# Autodesk Inventor assembly: DriveTrainAssembly
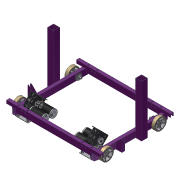
[picture p0: Inventor's stored thumbnail of the model, 180x180]
Saved by Autodesk Inventor 2012 (Build 160160000, 160)
## iProperties
Created: 2013-01-06
Part Number: DriveTrainAssembly
Document SubType Name: Assembly
Designer: JesseK
Mass: 18854.9 g
Surface Area: 24329.7 cm^2
Volume: 23563.9 cm^3
Density: 0.800159 g/cm^3
Author: JesseK
## Documents named in this file (15)
- Z:\UserData\Documents\Inventor\team1885frc\Robot2013\DriveTrain\DriveTrainAssembly.iam
- Z:\UserData\Documents\Inventor\team1885frc\Robot2013\DriveTrain\DriveTrainFrameAssembly.iam
- Z:\UserData\Documents\Inventor\team1885frc\Robot2013\DriveTrain\WheelBearingBlock.ipt
- Z:\UserData\Documents\Inventor\team1885frc\Hardware\Bearings\500id_1.125od_hex_flange_bearing.ipt
- Z:\UserData\Documents\Inventor\team1885frc\Robot2013\DriveTrain\WheelAxle.ipt
- Z:\UserData\Documents\Inventor\team1885frc\AndyMark\4 Perf ThruTread 500 Hex.ipt
- Z:\UserData\Documents\Inventor\team1885frc\VEXPro\Gears\44T-0500-hex.217-2710.20121204.ipt
- Z:\UserData\Documents\Inventor\team1885frc\AndyMark\Sprocket_Num25_22T_0.5bore.ipt
- Z:\UserData\Documents\Inventor\team1885frc\VEXPro\Gearboxes\SingleSpeed_12x64\SingleSpeed_12x64.iam
- Z:\UserData\Documents\Inventor\team1885frc\VEXPro\Gears\30T-0500-hex.217-2705.20121204.ipt
- Z:\UserData\Documents\Inventor\team1885frc\Robot2013\DriveTrain\BumperRepresentation.ipt
- Z:\UserData\Documents\Inventor\team1885frc\Robot2013\DriveTrain\GearboxMountPlate.ipt
- Z:\UserData\Documents\Inventor\team1885frc\Robot2013\DriveTrain\GearboxMountSpacer.ipt
- Z:\UserData\Documents\Inventor\team1885frc\VEXPro\Gears\34T-0500-hex.217-2706.20121204.ipt
- Z:\UserData\Documents\Inventor\team1885frc\VEXPro\Gears\50T-0375-hex.217-2711.20121204.ipt
## Components (39 placed, 14 different names)
1. DriveTrainFrameAssembly:1 [sub-assembly] — Mate:16, Flush:8, Mate:79, Mate:80, Mate:81, Mate:82, Flush:20, Mate:86, Mate:88, Flush:23, Flush:24, Mate:94, Mate:95, Mate:98, Mate:99, Flush:25, Mate:101, Mate:112, Flush:26, Mate:114, Flush:29, Mate:115, Flush:30, Mate:116, Mate:121, Mate:122, Mate:126
2. WheelBearingBlock:2 — Mate:110, Mate:111, Mate:112, Flush:26, Flush:27, Flush:28
3. WheelBearingBlock:3 — Mate:114, Flush:29, Mate:117, Flush:31, Mate:118, Mate:126
4. 500id_1.125od_hex_flange_bearing:2 — Mate:109, Flush:32, Mate:124
5. 500id_1.125od_hex_flange_bearing:3 — Mate:33, Mate:111, Flush:27
6. 500id_1.125od_hex_flange_bearing:4 — Flush:8, Mate:118, Mate:119
7. 500id_1.125od_hex_flange_bearing:5 — Mate:16, Mate:72
8. 500id_1.125od_hex_flange_bearing:8 — Mate:42, Mate:45, Mate:120, Mate:123, Flush:34
9. 500id_1.125od_hex_flange_bearing:9 — Mate:46, Mate:117, Flush:31
10. 500id_1.125od_hex_flange_bearing:11 — Mate:76, Mate:108, Flush:33, Mate:125
11. 500id_1.125od_hex_flange_bearing:12 — Mate:110, Flush:28, Mate:113
12. WheelAxle:2 — Mate:36, Mate:37, Mate:63
13. WheelAxle:3 — Mate:32, Flush:12, Mate:34, Mate:58, Mate:61, Mate:113
14. WheelAxle:4 — Mate:47, Mate:48, Mate:58, Mate:59, Mate:119
15. WheelAxle:5 — Mate:42, Mate:49, Mate:50, Mate:67, Mate:68, Mate:123
16. 4 Perf ThruTread 500 Hex:1 — Mate:32, Mate:33, Flush:12, Mate:34
17. 4 Perf ThruTread 500 Hex:2 — Mate:36, Mate:37, Tangent:3, Mate:124, Mate:125
18. 4 Perf ThruTread 500 Hex:4 — Mate:46, Mate:47, Mate:48
19. 4 Perf ThruTread 500 Hex:5 — Mate:45, Mate:49, Mate:50
20. 44T-0500-hex.217-2710.20121204:1 — Mate:67, Mate:73, Flush:16
21. Sprocket_Num25_22T_0.5bore:1 — Mate:59, Flush:14
22. Sprocket_Num25_22T_0.5bore:2 — Mate:61, Flush:13
23. Sprocket_Num25_22T_0.5bore:3 — Mate:63, Flush:13, Mate:76, Mate:130, Mate:131
24. Sprocket_Num25_22T_0.5bore:4 — Mate:68, Flush:14, Mate:72, Mate:73
25. 30T-0500-hex.217-2705.20121204:1 — Flush:16, Mate:87
26. BumperRepresentation:1 — Mate:79, Mate:80, Mate:83, Tangent:3
27. BumperRepresentation:2 — Mate:81, Mate:82, Mate:83
28. SingleSpeed_12x64:2 [sub-assembly] — Mate:88, Mate:89, Tangent:1, Flush:35, Mate:129
29. SingleSpeed_12x64:3 [sub-assembly] — Flush:20, Mate:86, Mate:87, Mate:89, Mate:91, Tangent:2
30. GearboxMountPlate:1 — Flush:23, Flush:24, Mate:91, Mate:92, Mate:93, Tangent:2
31. GearboxMountSpacer:1 — Mate:92, Mate:94
32. GearboxMountSpacer:2 — Mate:93, Mate:95
33. GearboxMountSpacer:3 — Mate:99, Mate:100, Mate:128
34. GearboxMountSpacer:4 — Mate:98, Mate:127
35. GearboxMountPlate:2 — Flush:25, Mate:100, Mate:101, Tangent:1, Mate:127, Mate:128
36. WheelBearingBlock:4 — Mate:120, Mate:121, Mate:122, Flush:34
37. WheelBearingBlock:5 — Mate:108, Mate:109, Mate:115, Flush:30, Mate:116, Flush:32, Flush:33
38. 34T-0500-hex.217-2706.20121204:1 — Flush:35, Mate:129
39. 50T-0375-hex.217-2711.20121204:1 — Mate:130, Mate:131
## Relationships (86: Mate 64, Flush 19, Tangent 3)
- Mate:16: DriveTrainFrameAssembly:1 ↔ 500id_1.125od_hex_flange_bearing:5
- Flush:8: DriveTrainFrameAssembly:1 ↔ 500id_1.125od_hex_flange_bearing:4
- Mate:32: WheelAxle:3 ↔ 4 Perf ThruTread 500 Hex:1
- Mate:33 (4.7625 mm): 500id_1.125od_hex_flange_bearing:3 ↔ 4 Perf ThruTread 500 Hex:1
- Flush:12: WheelAxle:3 ↔ 4 Perf ThruTread 500 Hex:1
- Mate:34: WheelAxle:3 ↔ 4 Perf ThruTread 500 Hex:1
- Mate:36: WheelAxle:2 ↔ 4 Perf ThruTread 500 Hex:2
- Mate:37: WheelAxle:2 ↔ 4 Perf ThruTread 500 Hex:2
- Mate:42: 500id_1.125od_hex_flange_bearing:8 ↔ WheelAxle:5
- Mate:45 (3.175 mm): 500id_1.125od_hex_flange_bearing:8 ↔ 4 Perf ThruTread 500 Hex:5
- Mate:46 (6.35 mm): 500id_1.125od_hex_flange_bearing:9 ↔ 4 Perf ThruTread 500 Hex:4
- Mate:47: WheelAxle:4 ↔ 4 Perf ThruTread 500 Hex:4
- Mate:48: WheelAxle:4 ↔ 4 Perf ThruTread 500 Hex:4
- Mate:49: WheelAxle:5 ↔ 4 Perf ThruTread 500 Hex:5
- Mate:50: WheelAxle:5 ↔ 4 Perf ThruTread 500 Hex:5
- Mate:58: WheelAxle:3 ↔ WheelAxle:4
- Mate:59: WheelAxle:4 ↔ Sprocket_Num25_22T_0.5bore:1
- Mate:61: WheelAxle:3 ↔ Sprocket_Num25_22T_0.5bore:2
- Mate:63: WheelAxle:2 ↔ Sprocket_Num25_22T_0.5bore:3
- Mate:67: WheelAxle:5 ↔ 44T-0500-hex.217-2710.20121204:1
- Mate:68: WheelAxle:5 ↔ Sprocket_Num25_22T_0.5bore:4
- Flush:13: Sprocket_Num25_22T_0.5bore:2 ↔ Sprocket_Num25_22T_0.5bore:3
- Flush:14: Sprocket_Num25_22T_0.5bore:1 ↔ Sprocket_Num25_22T_0.5bore:4
- Mate:72: 500id_1.125od_hex_flange_bearing:5 ↔ Sprocket_Num25_22T_0.5bore:4
- Mate:73 (6.35 mm): 44T-0500-hex.217-2710.20121204:1 ↔ Sprocket_Num25_22T_0.5bore:4
- Flush:16: 44T-0500-hex.217-2710.20121204:1 ↔ 30T-0500-hex.217-2705.20121204:1
- Mate:76: 500id_1.125od_hex_flange_bearing:11 ↔ Sprocket_Num25_22T_0.5bore:3
- Mate:79: DriveTrainFrameAssembly:1 ↔ BumperRepresentation:1
- Mate:80: DriveTrainFrameAssembly:1 ↔ BumperRepresentation:1
- Mate:81: DriveTrainFrameAssembly:1 ↔ BumperRepresentation:2
- Mate:82: DriveTrainFrameAssembly:1 ↔ BumperRepresentation:2
- Mate:83: BumperRepresentation:1 ↔ BumperRepresentation:2
- Flush:20: DriveTrainFrameAssembly:1 ↔ SingleSpeed_12x64:3
- Mate:86: DriveTrainFrameAssembly:1 ↔ SingleSpeed_12x64:3
- Mate:87: 30T-0500-hex.217-2705.20121204:1 ↔ SingleSpeed_12x64:3
- Mate:88: DriveTrainFrameAssembly:1 ↔ SingleSpeed_12x64:2
- Mate:89: SingleSpeed_12x64:2 ↔ SingleSpeed_12x64:3
- Flush:23: DriveTrainFrameAssembly:1 ↔ GearboxMountPlate:1
- Flush:24: DriveTrainFrameAssembly:1 ↔ GearboxMountPlate:1
- Mate:91: SingleSpeed_12x64:3 ↔ GearboxMountPlate:1
- Mate:92: GearboxMountPlate:1 ↔ GearboxMountSpacer:1
- Mate:93: GearboxMountPlate:1 ↔ GearboxMountSpacer:2
- Mate:94: DriveTrainFrameAssembly:1 ↔ GearboxMountSpacer:1
- Mate:95: DriveTrainFrameAssembly:1 ↔ GearboxMountSpacer:2
- Mate:98: DriveTrainFrameAssembly:1 ↔ GearboxMountSpacer:4
- Mate:99: DriveTrainFrameAssembly:1 ↔ GearboxMountSpacer:3
- Flush:25: DriveTrainFrameAssembly:1 ↔ GearboxMountPlate:2
- Mate:100: GearboxMountSpacer:3 ↔ GearboxMountPlate:2
- Mate:101: DriveTrainFrameAssembly:1 ↔ GearboxMountPlate:2
- Tangent:1: SingleSpeed_12x64:2 ↔ GearboxMountPlate:2
- Tangent:2: SingleSpeed_12x64:3 ↔ GearboxMountPlate:1
- Tangent:3 (-50.8 mm): 4 Perf ThruTread 500 Hex:2 ↔ BumperRepresentation:1
- Mate:108: 500id_1.125od_hex_flange_bearing:11 ↔ WheelBearingBlock:5
- Mate:109: 500id_1.125od_hex_flange_bearing:2 ↔ WheelBearingBlock:5
- Mate:110: WheelBearingBlock:2 ↔ 500id_1.125od_hex_flange_bearing:12
- Mate:111: WheelBearingBlock:2 ↔ 500id_1.125od_hex_flange_bearing:3
- Mate:112: DriveTrainFrameAssembly:1 ↔ WheelBearingBlock:2
- Flush:26: DriveTrainFrameAssembly:1 ↔ WheelBearingBlock:2
- Flush:27: WheelBearingBlock:2 ↔ 500id_1.125od_hex_flange_bearing:3
- Flush:28: WheelBearingBlock:2 ↔ 500id_1.125od_hex_flange_bearing:12
- Mate:113: 500id_1.125od_hex_flange_bearing:12 ↔ WheelAxle:3
- Mate:114: DriveTrainFrameAssembly:1 ↔ WheelBearingBlock:3
- Flush:29: DriveTrainFrameAssembly:1 ↔ WheelBearingBlock:3
- Mate:115: DriveTrainFrameAssembly:1 ↔ WheelBearingBlock:5
- Flush:30: DriveTrainFrameAssembly:1 ↔ WheelBearingBlock:5
- Mate:116: DriveTrainFrameAssembly:1 ↔ WheelBearingBlock:5
- Mate:117: WheelBearingBlock:3 ↔ 500id_1.125od_hex_flange_bearing:9
- Flush:31: WheelBearingBlock:3 ↔ 500id_1.125od_hex_flange_bearing:9
- Mate:118: WheelBearingBlock:3 ↔ 500id_1.125od_hex_flange_bearing:4
- Mate:119: 500id_1.125od_hex_flange_bearing:4 ↔ WheelAxle:4
- Flush:32: 500id_1.125od_hex_flange_bearing:2 ↔ WheelBearingBlock:5
- Flush:33: 500id_1.125od_hex_flange_bearing:11 ↔ WheelBearingBlock:5
- Mate:120: 500id_1.125od_hex_flange_bearing:8 ↔ WheelBearingBlock:4
- Mate:121: DriveTrainFrameAssembly:1 ↔ WheelBearingBlock:4
- Mate:122: DriveTrainFrameAssembly:1 ↔ WheelBearingBlock:4
- Mate:123: 500id_1.125od_hex_flange_bearing:8 ↔ WheelAxle:5
- Flush:34: 500id_1.125od_hex_flange_bearing:8 ↔ WheelBearingBlock:4
- Mate:124 (6.35 mm): 500id_1.125od_hex_flange_bearing:2 ↔ 4 Perf ThruTread 500 Hex:2
- Mate:125: 500id_1.125od_hex_flange_bearing:11 ↔ 4 Perf ThruTread 500 Hex:2
- Mate:126: DriveTrainFrameAssembly:1 ↔ WheelBearingBlock:3
- Mate:127: GearboxMountSpacer:4 ↔ GearboxMountPlate:2
- Mate:128: GearboxMountSpacer:3 ↔ GearboxMountPlate:2
- Flush:35: SingleSpeed_12x64:2 ↔ 34T-0500-hex.217-2706.20121204:1
- Mate:129: SingleSpeed_12x64:2 ↔ 34T-0500-hex.217-2706.20121204:1
- Mate:130 (6.35 mm): Sprocket_Num25_22T_0.5bore:3 ↔ 50T-0375-hex.217-2711.20121204:1
- Mate:131: Sprocket_Num25_22T_0.5bore:3 ↔ 50T-0375-hex.217-2711.20121204:1
